# Autodesk Inventor assembly: Sweeper Model
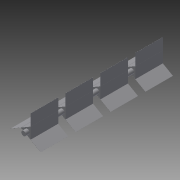
[picture p0: Inventor's stored thumbnail of the model, 180x180]
Saved by Autodesk Inventor 2014 (Build 180170000, 170)
## iProperties
Created: 2014-03-16
Part Number: Sweeper Model
Document SubType Name: Assembly
Designer: Pranav
Author: Pranav
## Documents named in this file (3)
- E:\Robotics Autodesk\Sweeper Model.iam
- E:\Robotics Autodesk\Sweeper Rod.ipt
- E:\Robotics Autodesk\Bush.iam
## Components (5 placed, 2 different names)
1. Sweeper Rod:1 — Rigid:1
2. Bush:1 [sub-assembly] — Rigid:1
3. Bush:2 [sub-assembly]
4. Bush:3 [sub-assembly]
5. Bush:4 [sub-assembly]
## Component patterns: (4 elements, first: Bush:1)
## Relationships (1: WeldJoint 1)
- Rigid:1 [WeldJoint] (-10.16 mm): Sweeper Rod:1 ↔ Bush:1
